# Autodesk Inventor assembly: FullSlideConnector
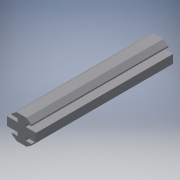
[picture p0: Inventor's stored thumbnail of the model, 180x180]
Saved by Autodesk Inventor 2017 (Build 210142000, 142)
## iProperties
Created: 2017-12-09
Part Number: FullSlideConnector
Document SubType Name: Assembly
Designer: User
Author: User
## Documents named in this file (2)
- C:\Robotics\CAD\2017-18_CAD\Prototypes\FullSlideConnector.iam
- C:\Robotics\CAD\2017-18_CAD\Prototypes\Sliderfor2020.ipt
## Components (2 placed, 1 different names)
1. Sliderfor2020:1 — Mate:1, Mate:2, Mate:3
2. Sliderfor2020:2 — Mate:1, Mate:2, Mate:3
## Relationships (3: Mate 3)
- Mate:1: Sliderfor2020:1 ↔ Sliderfor2020:2
- Mate:2: Sliderfor2020:1 ↔ Sliderfor2020:2
- Mate:3: Sliderfor2020:1 ↔ Sliderfor2020:2
